# Autodesk Inventor assembly: Wall Assembly
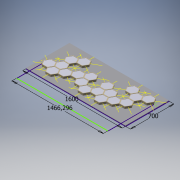
[picture p0: Inventor's stored thumbnail of the model, 180x180]
Saved by Autodesk Inventor 2019 (Build 230136000, 136)
## iProperties
Created: 2021-07-14
Part Number: Wall Assembly
Document SubType Name: Assembly
Designer: Lix
Author: Lix
## Documents named in this file (3)
- G:\Project\3d-printing\Models\My Own\Hexagonal Deco Lamp\Wall Assembly 160.iam
- G:\Project\3d-printing\Models\My Own\Hexagonal Deco Lamp\Wall - 160x70.ipt
- G:\Project\3d-printing\Models\My Own\Hexagonal Deco Lamp\Hexagonal Deco Lamp Assembly 150.iam
## Components (20 placed, 2 different names)
1. Wall - 160x70:1 — Mate:2, Mate:39
2. Hexagonal Deco Lamp Assembly 150:1 [sub-assembly] — Flush:1, Flush:2, Flush:3, Flush:4, Mate:3, Mate:4, Mate:13, Mate:14
3. Hexagonal Deco Lamp Assembly 150:2 [sub-assembly] — Flush:1, Mate:2, Mate:5, Mate:6, Mate:7, Mate:8, Mate:9, Mate:10
4. Hexagonal Deco Lamp Assembly 150:3 [sub-assembly] — Flush:2, Mate:3, Mate:4, Mate:5, Mate:6
5. Hexagonal Deco Lamp Assembly 150:4 [sub-assembly] — Flush:3, Flush:6, Mate:11, Mate:12
6. Hexagonal Deco Lamp Assembly 150:5 [sub-assembly] — Flush:5, Mate:9, Mate:10, Mate:11, Mate:12
7. Hexagonal Deco Lamp Assembly 150:6 [sub-assembly] — Flush:4, Flush:5, Mate:7, Mate:8
8. Hexagonal Deco Lamp Assembly 150:7 [sub-assembly] — Flush:6, Flush:7, Flush:9, Mate:13, Mate:14, Mate:15, Mate:16, Mate:17, Mate:18
9. Hexagonal Deco Lamp Assembly 150:8 [sub-assembly] — Flush:7, Flush:8, Flush:9, Mate:15, Mate:16
10. Hexagonal Deco Lamp Assembly 150:9 [sub-assembly] — Flush:8, Flush:10, Mate:17, Mate:18, Mate:19, Mate:20
11. Hexagonal Deco Lamp Assembly 150:10 [sub-assembly] — Flush:11, Flush:12, Mate:21, Mate:22, Mate:23, Mate:24, Mate:25, Mate:26, Mate:27, Mate:28
12. Hexagonal Deco Lamp Assembly 150:11 [sub-assembly] — Flush:13, Flush:14, Flush:15, Mate:23, Mate:24, Mate:29, Mate:30
13. Hexagonal Deco Lamp Assembly 150:12 [sub-assembly] — Flush:15, Flush:16, Mate:29, Mate:30, Mate:31, Mate:32
14. Hexagonal Deco Lamp Assembly 150:13 [sub-assembly] — Flush:14, Mate:27, Mate:28
15. Hexagonal Deco Lamp Assembly 150:14 [sub-assembly] — Flush:10, Flush:11, Mate:19, Mate:20, Mate:21, Mate:22
16. Hexagonal Deco Lamp Assembly 150:15 [sub-assembly] — Flush:12, Flush:13, Mate:25, Mate:26
17. Hexagonal Deco Lamp Assembly 150:16 [sub-assembly] — Flush:16, Flush:17, Flush:18, Mate:31, Mate:32, Mate:33, Mate:34
18. Hexagonal Deco Lamp Assembly 150:17 [sub-assembly] — Flush:17, Flush:18, Flush:19, Mate:33, Mate:34, Mate:35, Mate:36, Mate:37, Mate:38
19. Hexagonal Deco Lamp Assembly 150:18 [sub-assembly] — Flush:19, Mate:35, Mate:36
20. Hexagonal Deco Lamp Assembly 150:19 [sub-assembly] — Mate:37, Mate:38, Mate:39
## Relationships (57: Mate 38, Flush 19)
- Flush:1: Hexagonal Deco Lamp Assembly 150:1 ↔ Hexagonal Deco Lamp Assembly 150:2
- Flush:2: Hexagonal Deco Lamp Assembly 150:1 ↔ Hexagonal Deco Lamp Assembly 150:3
- Flush:3: Hexagonal Deco Lamp Assembly 150:1 ↔ Hexagonal Deco Lamp Assembly 150:4
- Flush:4: Hexagonal Deco Lamp Assembly 150:1 ↔ Hexagonal Deco Lamp Assembly 150:6
- Flush:5: Hexagonal Deco Lamp Assembly 150:5 ↔ Hexagonal Deco Lamp Assembly 150:6
- Flush:6: Hexagonal Deco Lamp Assembly 150:4 ↔ Hexagonal Deco Lamp Assembly 150:7
- Flush:7: Hexagonal Deco Lamp Assembly 150:7 ↔ Hexagonal Deco Lamp Assembly 150:8
- Flush:8: Hexagonal Deco Lamp Assembly 150:8 ↔ Hexagonal Deco Lamp Assembly 150:9
- Flush:9: Hexagonal Deco Lamp Assembly 150:7 ↔ Hexagonal Deco Lamp Assembly 150:8
- Flush:10: Hexagonal Deco Lamp Assembly 150:9 ↔ Hexagonal Deco Lamp Assembly 150:14
- Flush:11: Hexagonal Deco Lamp Assembly 150:10 ↔ Hexagonal Deco Lamp Assembly 150:14
- Flush:12: Hexagonal Deco Lamp Assembly 150:10 ↔ Hexagonal Deco Lamp Assembly 150:15
- Flush:13: Hexagonal Deco Lamp Assembly 150:11 ↔ Hexagonal Deco Lamp Assembly 150:15
- Flush:14: Hexagonal Deco Lamp Assembly 150:11 ↔ Hexagonal Deco Lamp Assembly 150:13
- Flush:15: Hexagonal Deco Lamp Assembly 150:11 ↔ Hexagonal Deco Lamp Assembly 150:12
- Flush:16: Hexagonal Deco Lamp Assembly 150:12 ↔ Hexagonal Deco Lamp Assembly 150:16
- Flush:17: Hexagonal Deco Lamp Assembly 150:16 ↔ Hexagonal Deco Lamp Assembly 150:17
- Flush:18: Hexagonal Deco Lamp Assembly 150:16 ↔ Hexagonal Deco Lamp Assembly 150:17
- Flush:19: Hexagonal Deco Lamp Assembly 150:17 ↔ Hexagonal Deco Lamp Assembly 150:18
- Mate:2: Wall - 160x70:1 ↔ Hexagonal Deco Lamp Assembly 150:2
- Mate:3: Hexagonal Deco Lamp Assembly 150:1 ↔ Hexagonal Deco Lamp Assembly 150:3
- Mate:4: Hexagonal Deco Lamp Assembly 150:1 ↔ Hexagonal Deco Lamp Assembly 150:3
- Mate:5: Hexagonal Deco Lamp Assembly 150:2 ↔ Hexagonal Deco Lamp Assembly 150:3
- Mate:6: Hexagonal Deco Lamp Assembly 150:2 ↔ Hexagonal Deco Lamp Assembly 150:3
- Mate:7: Hexagonal Deco Lamp Assembly 150:2 ↔ Hexagonal Deco Lamp Assembly 150:6
- Mate:8: Hexagonal Deco Lamp Assembly 150:2 ↔ Hexagonal Deco Lamp Assembly 150:6
- Mate:9: Hexagonal Deco Lamp Assembly 150:2 ↔ Hexagonal Deco Lamp Assembly 150:5
- Mate:10: Hexagonal Deco Lamp Assembly 150:2 ↔ Hexagonal Deco Lamp Assembly 150:5
- Mate:11: Hexagonal Deco Lamp Assembly 150:4 ↔ Hexagonal Deco Lamp Assembly 150:5
- Mate:12: Hexagonal Deco Lamp Assembly 150:4 ↔ Hexagonal Deco Lamp Assembly 150:5
- Mate:13: Hexagonal Deco Lamp Assembly 150:1 ↔ Hexagonal Deco Lamp Assembly 150:7
- Mate:14: Hexagonal Deco Lamp Assembly 150:1 ↔ Hexagonal Deco Lamp Assembly 150:7
- Mate:15: Hexagonal Deco Lamp Assembly 150:7 ↔ Hexagonal Deco Lamp Assembly 150:8
- Mate:16: Hexagonal Deco Lamp Assembly 150:7 ↔ Hexagonal Deco Lamp Assembly 150:8
- Mate:17: Hexagonal Deco Lamp Assembly 150:7 ↔ Hexagonal Deco Lamp Assembly 150:9
- Mate:18: Hexagonal Deco Lamp Assembly 150:7 ↔ Hexagonal Deco Lamp Assembly 150:9
- Mate:19: Hexagonal Deco Lamp Assembly 150:9 ↔ Hexagonal Deco Lamp Assembly 150:14
- Mate:20: Hexagonal Deco Lamp Assembly 150:9 ↔ Hexagonal Deco Lamp Assembly 150:14
- Mate:21: Hexagonal Deco Lamp Assembly 150:10 ↔ Hexagonal Deco Lamp Assembly 150:14
- Mate:22: Hexagonal Deco Lamp Assembly 150:10 ↔ Hexagonal Deco Lamp Assembly 150:14
- Mate:23: Hexagonal Deco Lamp Assembly 150:10 ↔ Hexagonal Deco Lamp Assembly 150:11
- Mate:24: Hexagonal Deco Lamp Assembly 150:10 ↔ Hexagonal Deco Lamp Assembly 150:11
- Mate:25: Hexagonal Deco Lamp Assembly 150:10 ↔ Hexagonal Deco Lamp Assembly 150:15
- Mate:26: Hexagonal Deco Lamp Assembly 150:10 ↔ Hexagonal Deco Lamp Assembly 150:15
- Mate:27: Hexagonal Deco Lamp Assembly 150:10 ↔ Hexagonal Deco Lamp Assembly 150:13
- Mate:28: Hexagonal Deco Lamp Assembly 150:10 ↔ Hexagonal Deco Lamp Assembly 150:13
- Mate:29: Hexagonal Deco Lamp Assembly 150:11 ↔ Hexagonal Deco Lamp Assembly 150:12
- Mate:30: Hexagonal Deco Lamp Assembly 150:11 ↔ Hexagonal Deco Lamp Assembly 150:12
- Mate:31: Hexagonal Deco Lamp Assembly 150:12 ↔ Hexagonal Deco Lamp Assembly 150:16
- Mate:32: Hexagonal Deco Lamp Assembly 150:12 ↔ Hexagonal Deco Lamp Assembly 150:16
- Mate:33: Hexagonal Deco Lamp Assembly 150:16 ↔ Hexagonal Deco Lamp Assembly 150:17
- Mate:34: Hexagonal Deco Lamp Assembly 150:16 ↔ Hexagonal Deco Lamp Assembly 150:17
- Mate:35: Hexagonal Deco Lamp Assembly 150:17 ↔ Hexagonal Deco Lamp Assembly 150:18
- Mate:36: Hexagonal Deco Lamp Assembly 150:17 ↔ Hexagonal Deco Lamp Assembly 150:18
- Mate:37: Hexagonal Deco Lamp Assembly 150:17 ↔ Hexagonal Deco Lamp Assembly 150:19
- Mate:38: Hexagonal Deco Lamp Assembly 150:17 ↔ Hexagonal Deco Lamp Assembly 150:19
- Mate:39: Wall - 160x70:1 ↔ Hexagonal Deco Lamp Assembly 150:19
